# Autodesk Inventor assembly: uMule-komplet
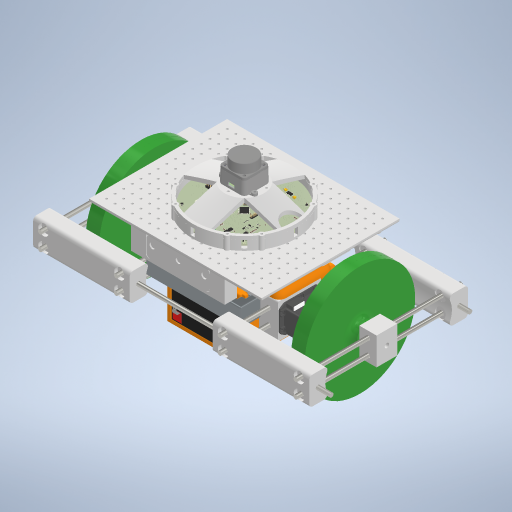
[picture p0: Inventor's stored thumbnail of the model, 512x512]
Saved by Autodesk Inventor 2024.3 (Build 283343000, 343)
## iProperties
Created: 2024-10-21
Part Number: uMule-komplet
Document SubType Name: Assembly
Designer: owozn
Author: owozn
## Documents named in this file (10)
- C:\Users\owozn\Documents\Nauka\Studia\mgr\Semestr_3\Magisterka\uMule\mechanics\uMule-komplet.iam
- C:\Users\owozn\Documents\Nauka\Studia\mgr\Semestr_3\Magisterka\uMule\mechanics\subsets\wheel\uMule-wheel_complete.iam
- C:\Users\owozn\Documents\Nauka\Studia\mgr\Semestr_3\Magisterka\uMule\mechanics\subsets\power_pack\uMule-power_pack.iam
- C:\Users\owozn\Documents\Nauka\Studia\mgr\Semestr_3\Magisterka\uMule\mechanics\subsets\long_frame_rod.ipt
- C:\Users\owozn\Documents\Nauka\Studia\mgr\Semestr_3\Magisterka\uMule\mechanics\subsets\attachments\hub\attachments_hub.ipt
- C:\Users\owozn\Documents\Nauka\Studia\mgr\Semestr_3\Magisterka\uMule\mechanics\subsets\attachments\raspberry_pi\RPI_assembly.iam
- C:\Users\owozn\Documents\Nauka\Studia\mgr\Semestr_3\Magisterka\uMule\mechanics\subsets\attachments\camera\camera_holder.ipt
- C:\Users\owozn\Documents\Nauka\Studia\mgr\Semestr_3\Magisterka\uMule\mechanics\subsets\attachments\main_board\main_board.iam
- C:\Users\owozn\Documents\Nauka\Studia\mgr\Semestr_3\Magisterka\uMule\mechanics\subsets\attachments\camera\camera_model.ipt
- C:\Users\owozn\Documents\Nauka\Studia\mgr\Semestr_3\Magisterka\uMule\mechanics\subsets\ball_caster_full.iam
## Components (11 placed, 9 different names)
1. uMule-wheel_complete:1 [sub-assembly] — Mate:5, Flush:2, Flush:3, Flush:4, Mate:8, Flush:13, Mate:9, Flush:15, Mate:10, Mate:38
2. uMule-wheel_complete:2 [sub-assembly] — Mate:5, Flush:2, Flush:3, Mate:7
3. uMule-power_pack:1 [sub-assembly] — Mate:7, Flush:4, Mate:8, Flush:16, Flush:17, Mate:13, Flush:18, Mate:36
4. long_frame_rod:1 — Flush:13, Mate:10
5. long_frame_rod:2 — Mate:9, Flush:15, Mate:40
6. attachments_hub:1 — Flush:16, Flush:17, Mate:11, Mate:13, Flush:18, Mate:18, Mate:27, Mate:28, Mate:29, Mate:30, Mate:33, Mate:34, Mate:35, Mate:37
7. RPI_assembly:1 [sub-assembly] — Mate:11, Mate:28, Mate:29
8. camera_holder:1 — Mate:31, Mate:32, Flush:19, Mate:33, Mate:34, Mate:35
9. main_board:1 [sub-assembly] — Mate:18, Mate:27, Mate:30, Mate:39
10. camera_model:1 — Mate:31, Mate:32, Flush:19
11. ball_caster_full:1 [sub-assembly] — Mate:36, Mate:37
## Relationships (31: Mate 22, Flush 9)
- Mate:5 (278 mm): uMule-wheel_complete:1 ↔ uMule-wheel_complete:2
- Flush:2: uMule-wheel_complete:1 ↔ uMule-wheel_complete:2
- Flush:3: uMule-wheel_complete:1 ↔ uMule-wheel_complete:2
- Mate:7 (6.5 mm): uMule-wheel_complete:2 ↔ uMule-power_pack:1
- Flush:4: uMule-wheel_complete:1 ↔ uMule-power_pack:1
- Mate:8 (4 mm): uMule-wheel_complete:1 ↔ uMule-power_pack:1
- Flush:13 (-4 mm): uMule-wheel_complete:1 ↔ long_frame_rod:1
- Mate:9: uMule-wheel_complete:1 ↔ long_frame_rod:2
- Flush:15: uMule-wheel_complete:1 ↔ long_frame_rod:2
- Mate:10: uMule-wheel_complete:1 ↔ long_frame_rod:1
- Flush:16: uMule-power_pack:1 ↔ attachments_hub:1
- Flush:17: uMule-power_pack:1 ↔ attachments_hub:1
- Mate:11: attachments_hub:1 ↔ RPI_assembly:1
- Mate:13: uMule-power_pack:1 ↔ attachments_hub:1
- Flush:18: uMule-power_pack:1 ↔ attachments_hub:1
- Mate:18: attachments_hub:1 ↔ main_board:1
- Mate:27: attachments_hub:1 ↔ main_board:1
- Mate:28: attachments_hub:1 ↔ RPI_assembly:1
- Mate:29: attachments_hub:1 ↔ RPI_assembly:1
- Mate:30: attachments_hub:1 ↔ main_board:1
- Mate:31: camera_holder:1 ↔ camera_model:1
- Mate:32: camera_holder:1 ↔ camera_model:1
- Flush:19: camera_holder:1 ↔ camera_model:1
- Mate:33: attachments_hub:1 ↔ camera_holder:1
- Mate:34: attachments_hub:1 ↔ camera_holder:1
- Mate:35: attachments_hub:1 ↔ camera_holder:1
- Mate:36: uMule-power_pack:1 ↔ ball_caster_full:1
- Mate:37: attachments_hub:1 ↔ ball_caster_full:1
- Mate:38: uMule-wheel_complete:1
- Mate:39: main_board:1
- Mate:40: long_frame_rod:2
